# Autodesk Inventor assembly: Ball Screw Assembly
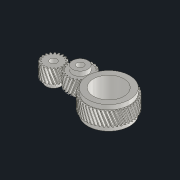
[picture p0: Inventor's stored thumbnail of the model, 180x180]
Saved by Autodesk Inventor 2021 (Build 250183000, 183)
## iProperties
Created: 2020-10-12
Part Number: Ball Screw Assembly
Document SubType Name: Assembly
Designer: Eugene Tang
Mass: 11976.1 g
Surface Area: 10762 cm^2
Volume: 3746.88 cm^3
Density: 3.19629 g/cm^3
Author: Eugene Tang
## Documents named in this file (20)
- C:\Users\teuge\OneDrive - Curtin University of Technology Australia\Y4S2\DFM\Group Project\CAD\Master\Ball Screw Assembly.iam
- C:\Users\teuge\OneDrive - Curtin University of Technology Australia\Y4S2\DFM\Group Project\CAD\Master\Screw.ipt
- C:\Users\teuge\OneDrive - Curtin University of Technology Australia\Y4S2\DFM\Group Project\CAD\Master\Steering Gear.ipt
- C:\Users\teuge\OneDrive - Curtin University of Technology Australia\Y4S2\DFM\Group Project\CAD\Parts\Involute Spline\Involute Spline Connection1.iam
- C:\Users\teuge\OneDrive - Curtin University of Technology Australia\Y4S2\DFM\Group Project\CAD\Master\Shell.ipt
- C:\Users\teuge\OneDrive - Curtin University of Technology Australia\Y4S2\DFM\Group Project\CAD\Parts\Assemblies\Bearing1.iam
- C:\Users\teuge\OneDrive - Curtin University of Technology Australia\Y4S2\DFM\Group Project\CAD\Parts\Gears\Spur Gears2.iam
- C:\Users\teuge\OneDrive - Curtin University of Technology Australia\Y4S2\DFM\Group Project\CAD\Parts\Gears\Spur Gears3.iam
- C:\Users\teuge\OneDrive - Curtin University of Technology Australia\Y4S2\DFM\Group Project\CAD\Master\Ball Screw Nut 1.0.ipt
- C:\Users\teuge\OneDrive - Curtin University of Technology Australia\Y4S2\DFM\Group Project\CAD\Parts\Assemblies\Bearing2.iam
- C:\Users\teuge\OneDrive - Curtin University of Technology Australia\Y4S2\DFM\Group Project\CAD\Master\Ball Screw Assembly\Design Accelerator\Bearing3.iam
- C:\Users\teuge\OneDrive - Curtin University of Technology Australia\Y4S2\DFM\Group Project\CAD\Parts\Gears\Spur Gears7.iam
- C:\Users\teuge\OneDrive - Curtin University of Technology Australia\Y4S2\DFM\Group Project\CAD\Parts\Gear Pins.ipt
- C:\Users\teuge\OneDrive - Curtin University of Technology Australia\Y4S2\DFM\Group Project\CAD\Parts\Gears\Spur Gear12.ipt
- C:\Users\teuge\OneDrive - Curtin University of Technology Australia\Y4S2\DFM\Group Project\CAD\Master\Ball Screw Assembly\Design Accelerator\Bearing6.iam
- C:\Users\teuge\OneDrive - Curtin University of Technology Australia\Y4S2\DFM\Group Project\CAD\Parts\Assemblies\Bearing7.iam
- C:\Users\teuge\OneDrive - Curtin University of Technology Australia\Y4S2\DFM\Group Project\CAD\Master\Steering Shaft.ipt
- C:\Users\teuge\OneDrive - Curtin University of Technology Australia\Y4S2\DFM\Group Project\CAD\Parts\Assemblies\Tie Rod Assembly.iam
- C:\Users\teuge\OneDrive - Curtin University of Technology Australia\Y4S2\DFM\Group Project\CAD\Parts\Assemblies\Motor Assembly.iam
- E:\Y4S2\DFM\Group Project\Parameters.xlsx
## Components (17 placed, 10 different names)
1. Screw:1 — Mate:14, Mate:18, Mate:79, Mate:99, Mate:100, Mate:101, Mate:102, Mate:103, Flush:22
2. Steering Gear:1 — Mate:14, Mate:18, Mate:96, Mate:97
3. Involute Spline Connection:1 [sub-assembly]
4. Bearing:1 [sub-assembly] — Mate:98, Flush:21
5. Spur Gears:1 [sub-assembly] — Flush:5, Flush:7
6. Spur Gears:2 [sub-assembly] — Mate:78, Flush:6, Mate:104, Flush:23
7. Bearing:2 [sub-assembly]
8. Bearing:3 [sub-assembly]
9. Spur Gears:3 [sub-assembly] — Flush:5, Mate:80, Flush:7
10. Gear Pins:1 — Mate:78, Flush:6, Mate:79, Mate:80, Mate:89, Flush:17, Mate:90, Mate:91
11. Bearing:6 [sub-assembly] — Mate:89, Flush:17
12. Bearing:7 [sub-assembly] — Mate:90, Mate:91
13. Steering Shaft:1 — Mate:96, Mate:97, Mate:98, Flush:21
14. Tie Rod Assembly:1 [sub-assembly] — Mate:99, Mate:101, Flush:22
15. Tie Rod Assembly:2 [sub-assembly] — Mate:100, Mate:102, Mate:103
16. Motor Assembly:2 [sub-assembly] — Mate:104, Flush:23
17. Shell:1
## Relationships (24: Mate 17, Flush 7)
- Mate:14: Screw:1 ↔ Steering Gear:1
- Mate:18 (-22.5 mm): Screw:1 ↔ Steering Gear:1
- Flush:5: Spur Gears:1 ↔ Spur Gears:3
- Mate:78: Spur Gears:2 ↔ Gear Pins:1
- Flush:6: Spur Gears:2 ↔ Gear Pins:1
- Mate:79: Screw:1 ↔ Gear Pins:1
- Mate:80: Spur Gears:3 ↔ Gear Pins:1
- Flush:7: Spur Gears:1 ↔ Spur Gears:3
- Mate:89: Gear Pins:1 ↔ Bearing:6
- Flush:17: Gear Pins:1 ↔ Bearing:6
- Mate:90: Gear Pins:1 ↔ Bearing:7
- Mate:91: Gear Pins:1 ↔ Bearing:7
- Mate:96: Steering Gear:1 ↔ Steering Shaft:1
- Mate:97: Steering Gear:1 ↔ Steering Shaft:1
- Mate:98: Bearing:1 ↔ Steering Shaft:1
- Flush:21: Bearing:1 ↔ Steering Shaft:1
- Mate:99: Screw:1 ↔ Tie Rod Assembly:1
- Mate:100: Screw:1 ↔ Tie Rod Assembly:2
- Mate:101: Screw:1 ↔ Tie Rod Assembly:1
- Mate:102: Screw:1 ↔ Tie Rod Assembly:2
- Mate:103: Screw:1 ↔ Tie Rod Assembly:2
- Flush:22: Screw:1 ↔ Tie Rod Assembly:1
- Mate:104: Spur Gears:2 ↔ Motor Assembly:2
- Flush:23: Spur Gears:2 ↔ Motor Assembly:2
## Named parameters: TD = 0.5, Ball_DIA = 6.35 mm, Screw_L = 292 mm, Screw_DIA = 36 mm, Screw_PITCH = 1 mm, Screw_LEAD = 10 mm, Nut_L = 80 mm, Nut_OD = 66 mm, Flange_OFFSET = 50 mm, Flange_DIA = 80 mm, Flange_L = 10 mm, BPath_REVQ = 5.75, Tread_OFFSET = 8.075 mm, TotalSteeringColumn_L = 840 mm, FSteeringColumn_L = 100 mm, RSteeringColumn_L = 80 mm, SteeringColumnChamfer_DEG = 20 deg, Rack_L = 307.252 mm, SteeringColumn_DIA = 26 mm, contact = 26 mm, rack_DEPTH = 6 mm, ToothH = 5.62 mm, SteererGearPlane = 18.76 mm, GearLength = 45 mm, NutCapTread_L = 25 mm, NutCapTread_THICKNESS = 4.5 mm, NutCap_OD = 60 mm, Gear_Thickness = 50 mm, GearToHub_Ratio = 0.6, GearThickness = 50 mm, GeartoHub_Ratio = 0.6, Facewidth = 30 mm, Tread_OD = 45 mm, Hub_L = 10 mm, SupportFlange_THICKNESS = 5 mm, GearKey_L = 40 mm, PinionKey_L = 20 mm, IntermediateKey_L = 20 mm
